# Autodesk Inventor assembly: BG_Tretboot_Rumpf
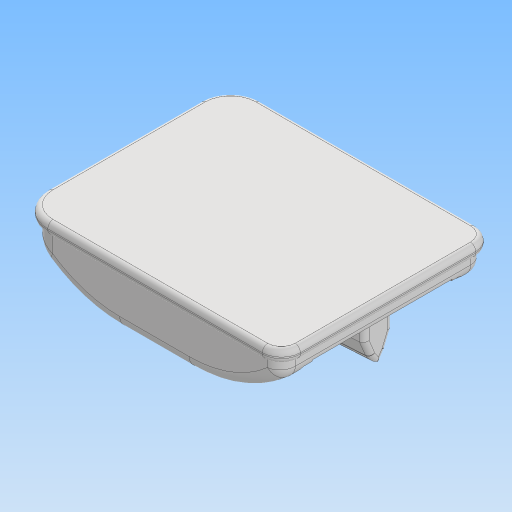
[picture p0: Inventor's stored thumbnail of the model, 512x512]
Saved by Autodesk Inventor 2024.4 (Build 284460000, 460)
## iProperties
Created: 2026-01-17
Part Number: BG_Tretboot_Rumpf
Document SubType Name: Assembly
Designer: windows-desktop
Mass: 877795 g
Surface Area: 123445 cm^2
Volume: 877795 cm^3
Density: 1 g/cm^3
Author: windows-desktop
## Documents named in this file (3)
- C:\Users\windows-desktop\Desktop\Studium\Konstruktion\VaultWorkspace\Daten\I60-Konstruktion\I60-Gruppe-4\Bluhm\BG_Tretboot_Rumpf.iam
- C:\Users\windows-desktop\Desktop\Studium\Konstruktion\VaultWorkspace\Daten\I60-Konstruktion\I60-Gruppe-4\Bluhm\Rumpf_Deck_Verbindungsstück.ipt
- C:\Users\windows-desktop\Desktop\Studium\Konstruktion\VaultWorkspace\Daten\I60-Konstruktion\I60-Gruppe-4\Bluhm\kurzer_Mittelrumpf_Version_02.ipt
## Components (2 placed, 2 different names)
1. Rumpf_Deck_Verbindungsstück:1 — Passend:1, Passend:2
2. kurzer_Mittelrumpf_Version_02:1 — Passend:1, Passend:2
## Relationships (2: Mate 2)
- Passend:1 [Mate]: Rumpf_Deck_Verbindungsstück:1 ↔ kurzer_Mittelrumpf_Version_02:1
- Passend:2 [Mate]: Rumpf_Deck_Verbindungsstück:1 ↔ kurzer_Mittelrumpf_Version_02:1
